# Autodesk Inventor assembly: Assembly1
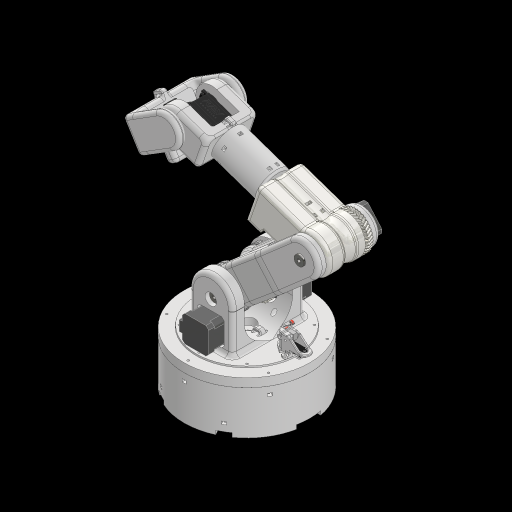
[picture p0: Inventor's stored thumbnail of the model, 512x512]
Saved by Autodesk Inventor 2023 (Build 270158000, 158)
## iProperties
Created: 2023-03-01
Part Number: Assembly1
Document SubType Name: Assembly
Designer: tandu
Author: tandu
## Documents named in this file (25)
- C:\Users\tandu\Documents\GrabCAD\Robotic Arm Project\IndustrialStyledVersion\V1\Assembly1.iam
- C:\Users\tandu\Documents\GrabCAD\Robotic Arm Project\IndustrialStyledVersion\V1\ParametersPart.ipt
- C:\Users\tandu\Documents\GrabCAD\Robotic Arm Project\IndustrialStyledVersion\V1\NEMA17-42A02C-Body.ipt
- C:\Users\tandu\Documents\GrabCAD\Robotic Arm Project\IndustrialStyledVersion\V1\Base.ipt
- C:\Users\tandu\Documents\GrabCAD\Robotic Arm Project\IndustrialStyledVersion\V1\BaseLid.ipt
- C:\Users\tandu\Documents\GrabCAD\Robotic Arm Project\IndustrialStyledVersion\V1\Assembly1\Design Accelerator\Spur Gears1.iam
- C:\Users\tandu\Documents\GrabCAD\Robotic Arm Project\IndustrialStyledVersion\V1\FirstLink.ipt
- C:\Users\tandu\Documents\GrabCAD\Robotic Arm Project\IndustrialStyledVersion\V1\92981A312_Alloy Steel Shoulder Screws.ipt
- C:\Users\tandu\Documents\GrabCAD\Robotic Arm Project\IndustrialStyledVersion\V1\4390N117_Flanged Ultra-Thin Ball Bearing.ipt
- C:\Users\tandu\Documents\GrabCAD\Robotic Arm Project\IndustrialStyledVersion\V1\Assembly1\Design Accelerator\Link1Gears.iam
- C:\Users\tandu\Documents\GrabCAD\Robotic Arm Project\IndustrialStyledVersion\V1\Assembly1\Design Accelerator\Link1Gear1.ipt
- C:\Users\tandu\Documents\GrabCAD\Robotic Arm Project\IndustrialStyledVersion\V1\Assembly1\Design Accelerator\Link1Gear2.ipt
- C:\Users\tandu\Documents\GrabCAD\Robotic Arm Project\IndustrialStyledVersion\V1\Assembly1\Design Accelerator\Link2 Gears1.iam
- C:\Users\tandu\Documents\GrabCAD\Robotic Arm Project\IndustrialStyledVersion\V1\Assembly1\Design Accelerator\Link2 Gear2.ipt
- C:\Users\tandu\Documents\GrabCAD\Robotic Arm Project\IndustrialStyledVersion\V1\Assembly1\Design Accelerator\Link2Gear1.ipt
- C:\Users\tandu\Documents\GrabCAD\Robotic Arm Project\IndustrialStyledVersion\V1\MG995 Servo.iam
- C:\Users\tandu\Documents\GrabCAD\Robotic Arm Project\IndustrialStyledVersion\V1\Link3.ipt
- C:\Users\tandu\Documents\GrabCAD\Robotic Arm Project\IndustrialStyledVersion\V1\Link4.ipt
- C:\Users\tandu\Documents\GrabCAD\Robotic Arm Project\IndustrialStyledVersion\V1\REV-41-1097.ipt
- C:\Users\tandu\Documents\GrabCAD\Robotic Arm Project\IndustrialStyledVersion\V1\Link5.ipt
- C:\Users\tandu\Documents\GrabCAD\Robotic Arm Project\IndustrialStyledVersion\V1\Link4 Servo Horn.ipt
- C:\Users\tandu\Documents\GrabCAD\Robotic Arm Project\IndustrialStyledVersion\V1\ClawMountingPlate.ipt
- C:\Users\tandu\Documents\GrabCAD\Robotic Arm Project\IndustrialStyledVersion\V1\Optical Endstop.iam
- C:\Users\tandu\Documents\GrabCAD\Robotic Arm Project\IndustrialStyledVersion\V1\Limit Switch KW12-3.iam
- C:\Users\tandu\Documents\GrabCAD\Robotic Arm Project\IndustrialStyledVersion\V1\FirstJointHomingMount.ipt
## Components (41 placed, 23 different names)
1. ParametersPart:1
2. Base:1 — Flush:1, Flush:2, Flush:3, Insert:1, Insert:3, Insert:4, Insert:5, Mate:1
3. BaseLid:1 — Insert:3, Insert:4, Mate:7
4. Spur Gears:1 [sub-assembly] — Mate:1, Insert:6, Mate:7
5. FirstLink:1 — Insert:6, Insert:15, Insert:16, Insert:17, Insert:18, Insert:19, Insert:20, Insert:21, Tangent:1, Mate:9, Mate:11, Angle:3, Mate:12, Mate:14, Mate:17
6. Link1 Gears:1 [sub-assembly]
7. Link1 Gear1:1 — Mate:4, Flush:4, Rotation:1
8. Link2 Gear2:1 — Insert:23, Flush:4, Rotation:1, Insert:24, Insert:25, Flush:5, Rotation:2, Insert:26, Insert:27, Insert:28, Mate:19, Mate:20, Mate:21
9. Link1 Gear1:2 — Mate:5, Flush:5, Rotation:2
10. Link2 Gears:1 [sub-assembly]
11. Link2 Gear2:2 — Insert:29, Flush:6, Rotation:3, Insert:31, Insert:32, Insert:42, Insert:43
12. Link2 Gear1:1 — Mate:6, Flush:6, Rotation:3
13. Link3:1 — Insert:35, Insert:46, Mate:18
14. Link4:1 — Insert:35, Insert:37, Insert:39, Insert:40, Insert:41, Insert:44, Insert:45, Mate:18
15. MG995 Servo:1 [sub-assembly] — Insert:32
16. MG995 Servo:2 [sub-assembly] — Insert:37
17. REV-41-1097:1 — Insert:44, Insert:45, Insert:47
18. REV-41-1097:2 — Insert:42, Insert:43
19. Link5:1 — Angle:1, Insert:49, Insert:50, Insert:51, Insert:52
20. Link4 Servo Horn:1 — Insert:47, Angle:1
21. REV-41-1097:3 — Insert:49, Insert:50
22. 4390N117_Flanged Ultra-Thin Ball Bearing:10 — Insert:51
23. ClawMountingPlate:1
24. Optical Endstop:1 [sub-assembly] — Tangent:1, Angle:2, Mate:9, Mate:13, Mate:15
25. Limit Switch KW12-3:1 [sub-assembly] — Mate:11, Angle:3, Mate:16
26. FirstJointHomingMount:1 — Mate:12, Mate:13, Mate:14, Mate:15, Mate:16
27. Limit Switch KW12-3:2 [sub-assembly] — Mate:19, Mate:20, Mate:21
28. NEMA17-42A02C-Body:1 — Insert:1, Insert:5
29. NEMA17-42A02C-Body:2 — Insert:17, Insert:18, Mate:4
30. NEMA17-42A02C-Body:3 — Insert:15, Insert:16, Mate:5, Angle:2
31. NEMA17-42A02C-Body:4 — Insert:24, Insert:25, Mate:6
32. 92981A312_Alloy Steel Shoulder Screws:2 — Insert:26
33. 4390N117_Flanged Ultra-Thin Ball Bearing:7 — Insert:40, Insert:52
34. 4390N117_Flanged Ultra-Thin Ball Bearing:8 — Insert:41
35. 4390N117_Flanged Ultra-Thin Ball Bearing:9 — Insert:39
36. 4390N117_Flanged Ultra-Thin Ball Bearing:3 — Insert:27
37. 4390N117_Flanged Ultra-Thin Ball Bearing:4 — Insert:28, Insert:29
38. 4390N117_Flanged Ultra-Thin Ball Bearing:6 — Insert:31, Insert:46
39. 92981A312_Alloy Steel Shoulder Screws:1 — Insert:19
40. 4390N117_Flanged Ultra-Thin Ball Bearing:1 — Insert:21, Insert:23
41. 4390N117_Flanged Ultra-Thin Ball Bearing:2 — Insert:20
## Relationships (66: Insert 36, Mate 17, Flush 6, RelateRotation 3, Angle 3, Tangent 1)
- Flush:1: Base:1
- Flush:2: Base:1
- Flush:3: Base:1
- Insert:1: Base:1 ↔ NEMA17-42A02C-Body:1
- Insert:3: Base:1 ↔ BaseLid:1
- Insert:4: Base:1 ↔ BaseLid:1
- Insert:5: Base:1 ↔ NEMA17-42A02C-Body:1
- Mate:1: Base:1 ↔ Spur Gears:1
- Insert:6: Spur Gears:1 ↔ FirstLink:1
- Insert:15: FirstLink:1 ↔ NEMA17-42A02C-Body:3
- Insert:16: FirstLink:1 ↔ NEMA17-42A02C-Body:3
- Insert:17: FirstLink:1 ↔ NEMA17-42A02C-Body:2
- Insert:18: FirstLink:1 ↔ NEMA17-42A02C-Body:2
- Insert:19: FirstLink:1 ↔ 92981A312_Alloy Steel Shoulder Screws:1
- Insert:20: FirstLink:1 ↔ 4390N117_Flanged Ultra-Thin Ball Bearing:2
- Insert:21: FirstLink:1 ↔ 4390N117_Flanged Ultra-Thin Ball Bearing:1
- Insert:23: Link2 Gear2:1 ↔ 4390N117_Flanged Ultra-Thin Ball Bearing:1
- Mate:4: Link1 Gear1:1 ↔ NEMA17-42A02C-Body:2
- Flush:4: Link1 Gear1:1 ↔ Link2 Gear2:1
- Rotation:1 [RelateRotation] (0.25 ul): Link1 Gear1:1 ↔ Link2 Gear2:1
- Insert:24: Link2 Gear2:1 ↔ NEMA17-42A02C-Body:4
- Insert:25: Link2 Gear2:1 ↔ NEMA17-42A02C-Body:4
- Mate:5: Link1 Gear1:2 ↔ NEMA17-42A02C-Body:3
- Flush:5: Link2 Gear2:1 ↔ Link1 Gear1:2
- Rotation:2 [RelateRotation] (0.25 ul): Link2 Gear2:1 ↔ Link1 Gear1:2
- Insert:26: Link2 Gear2:1 ↔ 92981A312_Alloy Steel Shoulder Screws:2
- Insert:27: Link2 Gear2:1 ↔ 4390N117_Flanged Ultra-Thin Ball Bearing:3
- Insert:28: Link2 Gear2:1 ↔ 4390N117_Flanged Ultra-Thin Ball Bearing:4
- Insert:29: Link2 Gear2:2 ↔ 4390N117_Flanged Ultra-Thin Ball Bearing:4
- Mate:6: Link2 Gear1:1 ↔ NEMA17-42A02C-Body:4
- Flush:6: Link2 Gear2:2 ↔ Link2 Gear1:1
- Rotation:3 [RelateRotation] (0.25 ul): Link2 Gear2:2 ↔ Link2 Gear1:1
- Insert:31: Link2 Gear2:2 ↔ 4390N117_Flanged Ultra-Thin Ball Bearing:6
- Insert:32: Link2 Gear2:2 ↔ MG995 Servo:1
- Insert:35: Link3:1 ↔ Link4:1
- Insert:37: Link4:1 ↔ MG995 Servo:2
- Insert:39: Link4:1 ↔ 4390N117_Flanged Ultra-Thin Ball Bearing:9
- Insert:40: Link4:1 ↔ 4390N117_Flanged Ultra-Thin Ball Bearing:7
- Insert:41: Link4:1 ↔ 4390N117_Flanged Ultra-Thin Ball Bearing:8
- Insert:42: Link2 Gear2:2 ↔ REV-41-1097:2
- Insert:43: Link2 Gear2:2 ↔ REV-41-1097:2
- Insert:44: Link4:1 ↔ REV-41-1097:1
- Insert:45: Link4:1 ↔ REV-41-1097:1
- Insert:46: Link3:1 ↔ 4390N117_Flanged Ultra-Thin Ball Bearing:6
- Insert:47: REV-41-1097:1 ↔ Link4 Servo Horn:1
- Angle:1 (180 deg): Link5:1 ↔ Link4 Servo Horn:1
- Insert:49: Link5:1 ↔ REV-41-1097:3
- Insert:50: Link5:1 ↔ REV-41-1097:3
- Insert:51: Link5:1 ↔ 4390N117_Flanged Ultra-Thin Ball Bearing:10
- Mate:7: BaseLid:1 ↔ Spur Gears:1
- Insert:52: Link5:1 ↔ 4390N117_Flanged Ultra-Thin Ball Bearing:7
- Tangent:1: FirstLink:1 ↔ Optical Endstop:1
- Angle:2 (0 deg): Optical Endstop:1 ↔ NEMA17-42A02C-Body:3
- Mate:9: FirstLink:1 ↔ Optical Endstop:1
- Mate:11: FirstLink:1 ↔ Limit Switch KW12-3:1
- Angle:3 (0 deg): FirstLink:1 ↔ Limit Switch KW12-3:1
- Mate:12: FirstLink:1 ↔ FirstJointHomingMount:1
- Mate:13: Optical Endstop:1 ↔ FirstJointHomingMount:1
- Mate:14: FirstLink:1 ↔ FirstJointHomingMount:1
- Mate:15: Optical Endstop:1 ↔ FirstJointHomingMount:1
- Mate:16: Limit Switch KW12-3:1 ↔ FirstJointHomingMount:1
- Mate:17: FirstLink:1
- Mate:18: Link3:1 ↔ Link4:1
- Mate:19: Link2 Gear2:1 ↔ Limit Switch KW12-3:2
- Mate:20: Link2 Gear2:1 ↔ Limit Switch KW12-3:2
- Mate:21: Link2 Gear2:1 ↔ Limit Switch KW12-3:2
